# Autodesk Inventor assembly: OmniWheel
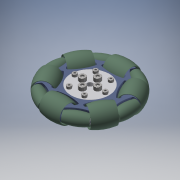
[picture p0: Inventor's stored thumbnail of the model, 180x180]
Saved by Autodesk Inventor 2019.1 (Build 231200000, 200)
## iProperties
Created: 2018-08-15
Part Number: OmniWheel
Material: Generisch
Document SubType Name: Assembly
Designer: JochenAlt
Author: JochenAlt
## Documents named in this file (9)
- D:\Projects\Ondine\CAD\OmniWheel.iam
- D:\Projects\Ondine\CAD\OmniWheel.ipt
- D:\Projects\Ondine\CAD\Mounting Hub.ipt
- C:\Users\JochenAlt\Documents\Inventor\Content Center Files\R2019\de-DE\DIN 912\DIN 912 - M3 x 0,5 x 8 x 6,75.ipt
- C:\Users\JochenAlt\Documents\Inventor\Content Center Files\R2019\de-DE\DIN 912\DIN 912 - M2 x 0,4 x 8 x 7.ipt
- C:\Users\JochenAlt\Documents\Inventor\Content Center Files\R2019\de-DE\DIN 934\DIN 934 - M2 x 0,4.ipt
- D:\Projects\Ondine\CAD\OmniWheelAxisSmall.ipt
- D:\Projects\Ondine\CAD\OmniWheelAxisBig.ipt
- D:\Projects\Ondine\CAD\Bearings\W 618_2 X.iam
## Components (54 placed, 8 different names)
1. OmniWheel:1 — Passend:1, Passend:2, Einfügen:1, Einfügen:2, Einfügen:3, Einfügen:4, Einfügen:5, Einfügen:6, Einfügen:7, Einfügen:8, Einfügen:9, Einfügen:10, Passend:4, Passend:6, Passend:8, Passend:10, Passend:12, Passend:14, Passend:15, Passend:16, Passend:17, Passend:18, Passend:19, Passend:20, Passend:21, Passend:23, Passend:24, Passend:25, Passend:26, Passend:27, Passend:28, Passend:29, Passend:30, Passend:31, Passend:32, Passend:33, Passend:34, Passend:35, Passend:36, Passend:37, Passend:38, Passend:39, Passend:64, Passend:65, Passend:66, Passend:67, Passend:68, Passend:69, Passend:70, Passend:71, Passend:72, Passend:73, Passend:74, Passend:75, Passend:76, Passend:77, Passend:78, Passend:79, Passend:80, Passend:81, Passend:82, Passend:83, Passend:84, Passend:85, Passend:86, Passend:87
2. Mounting Hub:1 — Passend:1, Passend:2
3. OmniWheelAxisSmall:1 — Passend:23, Passend:36, Passend:54, Passend:55
4. OmniWheelAxisSmall:2 — Passend:24, Passend:35, Passend:52, Passend:53
5. OmniWheelAxisSmall:3 — Passend:26, Passend:38, Passend:42, Passend:43
6. OmniWheelAxisSmall:4 — Passend:27, Passend:28, Passend:58, Passend:59
7. OmniWheelAxisSmall:5 — Passend:25, Passend:39, Passend:46, Passend:47
8. OmniWheelAxisSmall:6 — Passend:21, Passend:37, Passend:62, Passend:63
9. OmniWheelAxisBig:1 — Passend:15, Passend:31, Passend:60, Passend:61
10. OmniWheelAxisBig:2 — Passend:16, Passend:29, Passend:56, Passend:57
11. OmniWheelAxisBig:3 — Passend:19, Passend:33, Passend:44, Passend:45
12. OmniWheelAxisBig:4 — Passend:20, Passend:32, Passend:40, Passend:41
13. OmniWheelAxisBig:5 — Passend:17, Passend:30, Passend:50, Passend:51
14. OmniWheelAxisBig:6 — Passend:18, Passend:34, Passend:48, Passend:49
15. DIN 912 - ersetzt durch DIN EN ISO 4762 M3 x 8:1 — Einfügen:1
16. DIN 912 - ersetzt durch DIN EN ISO 4762 M3 x 8:2 — Einfügen:2
17. DIN 912 - ersetzt durch DIN EN ISO 4762 M3 x 8:3 — Einfügen:3
18. DIN 912 - ersetzt durch DIN EN ISO 4762 M3 x 8:4 — Einfügen:4
19. DIN 912 - ersetzt durch DIN EN ISO 4762 M2 x 8:1 — Einfügen:5, Passend:13
20. DIN 912 - ersetzt durch DIN EN ISO 4762 M2 x 8:2 — Einfügen:6, Passend:9
21. DIN 912 - ersetzt durch DIN EN ISO 4762 M2 x 8:3 — Einfügen:7, Passend:7
22. DIN 912 - ersetzt durch DIN EN ISO 4762 M2 x 8:4 — Einfügen:8, Passend:5
23. DIN 912 - ersetzt durch DIN EN ISO 4762 M2 x 8:5 — Einfügen:9, Passend:11
24. DIN 912 - ersetzt durch DIN EN ISO 4762 M2 x 8:6 — Einfügen:10, Passend:3
25. DIN 934 - ersetzt durch DIN EN 24032/28673/28674 M2:1 — Passend:3, Passend:4
26. DIN 934 - ersetzt durch DIN EN 24032/28673/28674 M2:2 — Passend:5, Passend:6
27. DIN 934 - ersetzt durch DIN EN 24032/28673/28674 M2:3 — Passend:7, Passend:8
28. DIN 934 - ersetzt durch DIN EN 24032/28673/28674 M2:4 — Passend:9, Passend:10
29. DIN 934 - ersetzt durch DIN EN 24032/28673/28674 M2:5 — Passend:11, Passend:12
30. DIN 934 - ersetzt durch DIN EN 24032/28673/28674 M2:6 — Passend:13, Passend:14
31. W 618_2 X:1 [sub-assembly] — Passend:41, Passend:64
32. W 618_2 X:2 [sub-assembly] — Passend:42, Passend:87
33. W 618_2 X:3 [sub-assembly] — Passend:40, Passend:65
34. W 618_2 X:4 [sub-assembly] — Passend:43, Passend:86
35. W 618_2 X:5 [sub-assembly] — Passend:44, Passend:85
36. W 618_2 X:6 [sub-assembly] — Passend:59, Passend:70
37. W 618_2 X:7 [sub-assembly] — Passend:58, Passend:71
38. W 618_2 X:8 [sub-assembly] — Passend:53, Passend:81
39. W 618_2 X:9 [sub-assembly] — Passend:52, Passend:80
40. W 618_2 X:10 [sub-assembly] — Passend:57, Passend:72
41. W 618_2 X:11 [sub-assembly] — Passend:51, Passend:76
42. W 618_2 X:12 [sub-assembly] — Passend:50, Passend:77
43. W 618_2 X:13 [sub-assembly] — Passend:54, Passend:75
44. W 618_2 X:14 [sub-assembly] — Passend:48, Passend:78
45. W 618_2 X:15 [sub-assembly] — Passend:49, Passend:79
46. W 618_2 X:16 [sub-assembly] — Passend:55, Passend:74
47. W 618_2 X:17 [sub-assembly] — Passend:56, Passend:73
48. W 618_2 X:18 [sub-assembly] — Passend:45, Passend:84
49. W 618_2 X:19 [sub-assembly] — Passend:46, Passend:82
50. W 618_2 X:20 [sub-assembly] — Passend:47, Passend:83
51. W 618_2 X:21 [sub-assembly] — Passend:60, Passend:69
52. W 618_2 X:22 [sub-assembly] — Passend:63, Passend:66
53. W 618_2 X:23 [sub-assembly] — Passend:62, Passend:67
54. W 618_2 X:24 [sub-assembly] — Passend:61, Passend:68
## Relationships (96: Mate 86, Insert 10)
- Passend:1 [Mate]: OmniWheel:1 ↔ Mounting Hub:1
- Passend:2 [Mate]: OmniWheel:1 ↔ Mounting Hub:1
- Einfügen:1 [Insert]: OmniWheel:1 ↔ DIN 912 - ersetzt durch DIN EN ISO 4762 M3 x 8:1
- Einfügen:2 [Insert]: OmniWheel:1 ↔ DIN 912 - ersetzt durch DIN EN ISO 4762 M3 x 8:2
- Einfügen:3 [Insert]: OmniWheel:1 ↔ DIN 912 - ersetzt durch DIN EN ISO 4762 M3 x 8:3
- Einfügen:4 [Insert]: OmniWheel:1 ↔ DIN 912 - ersetzt durch DIN EN ISO 4762 M3 x 8:4
- Einfügen:5 [Insert]: OmniWheel:1 ↔ DIN 912 - ersetzt durch DIN EN ISO 4762 M2 x 8:1
- Einfügen:6 [Insert]: OmniWheel:1 ↔ DIN 912 - ersetzt durch DIN EN ISO 4762 M2 x 8:2
- Einfügen:7 [Insert]: OmniWheel:1 ↔ DIN 912 - ersetzt durch DIN EN ISO 4762 M2 x 8:3
- Einfügen:8 [Insert]: OmniWheel:1 ↔ DIN 912 - ersetzt durch DIN EN ISO 4762 M2 x 8:4
- Einfügen:9 [Insert]: OmniWheel:1 ↔ DIN 912 - ersetzt durch DIN EN ISO 4762 M2 x 8:5
- Einfügen:10 [Insert]: OmniWheel:1 ↔ DIN 912 - ersetzt durch DIN EN ISO 4762 M2 x 8:6
- Passend:3 [Mate]: DIN 912 - ersetzt durch DIN EN ISO 4762 M2 x 8:6 ↔ DIN 934 - ersetzt durch DIN EN 24032/28673/28674 M2:1
- Passend:4 [Mate]: OmniWheel:1 ↔ DIN 934 - ersetzt durch DIN EN 24032/28673/28674 M2:1
- Passend:5 [Mate]: DIN 912 - ersetzt durch DIN EN ISO 4762 M2 x 8:4 ↔ DIN 934 - ersetzt durch DIN EN 24032/28673/28674 M2:2
- Passend:6 [Mate]: OmniWheel:1 ↔ DIN 934 - ersetzt durch DIN EN 24032/28673/28674 M2:2
- Passend:7 [Mate]: DIN 912 - ersetzt durch DIN EN ISO 4762 M2 x 8:3 ↔ DIN 934 - ersetzt durch DIN EN 24032/28673/28674 M2:3
- Passend:8 [Mate]: OmniWheel:1 ↔ DIN 934 - ersetzt durch DIN EN 24032/28673/28674 M2:3
- Passend:9 [Mate]: DIN 912 - ersetzt durch DIN EN ISO 4762 M2 x 8:2 ↔ DIN 934 - ersetzt durch DIN EN 24032/28673/28674 M2:4
- Passend:10 [Mate]: OmniWheel:1 ↔ DIN 934 - ersetzt durch DIN EN 24032/28673/28674 M2:4
- Passend:11 [Mate]: DIN 912 - ersetzt durch DIN EN ISO 4762 M2 x 8:5 ↔ DIN 934 - ersetzt durch DIN EN 24032/28673/28674 M2:5
- Passend:12 [Mate]: OmniWheel:1 ↔ DIN 934 - ersetzt durch DIN EN 24032/28673/28674 M2:5
- Passend:13 [Mate]: DIN 912 - ersetzt durch DIN EN ISO 4762 M2 x 8:1 ↔ DIN 934 - ersetzt durch DIN EN 24032/28673/28674 M2:6
- Passend:14 [Mate]: OmniWheel:1 ↔ DIN 934 - ersetzt durch DIN EN 24032/28673/28674 M2:6
- Passend:15 [Mate]: OmniWheel:1 ↔ OmniWheelAxisBig:1
- Passend:16 [Mate]: OmniWheel:1 ↔ OmniWheelAxisBig:2
- Passend:17 [Mate]: OmniWheel:1 ↔ OmniWheelAxisBig:5
- Passend:18 [Mate]: OmniWheel:1 ↔ OmniWheelAxisBig:6
- Passend:19 [Mate]: OmniWheel:1 ↔ OmniWheelAxisBig:3
- Passend:20 [Mate]: OmniWheel:1 ↔ OmniWheelAxisBig:4
- Passend:21 [Mate]: OmniWheel:1 ↔ OmniWheelAxisSmall:6
- Passend:23 [Mate]: OmniWheel:1 ↔ OmniWheelAxisSmall:1
- Passend:24 [Mate]: OmniWheel:1 ↔ OmniWheelAxisSmall:2
- Passend:25 [Mate]: OmniWheel:1 ↔ OmniWheelAxisSmall:5
- Passend:26 [Mate]: OmniWheel:1 ↔ OmniWheelAxisSmall:3
- Passend:27 [Mate]: OmniWheel:1 ↔ OmniWheelAxisSmall:4
- Passend:28 [Mate]: OmniWheel:1 ↔ OmniWheelAxisSmall:4
- Passend:29 [Mate] (-2 mm): OmniWheel:1 ↔ OmniWheelAxisBig:2
- Passend:30 [Mate] (2 mm): OmniWheel:1 ↔ OmniWheelAxisBig:5
- Passend:31 [Mate] (2 mm): OmniWheel:1 ↔ OmniWheelAxisBig:1
- Passend:32 [Mate] (2 mm): OmniWheel:1 ↔ OmniWheelAxisBig:4
- Passend:33 [Mate] (2 mm): OmniWheel:1 ↔ OmniWheelAxisBig:3
- Passend:34 [Mate] (2 mm): OmniWheel:1 ↔ OmniWheelAxisBig:6
- Passend:35 [Mate]: OmniWheel:1 ↔ OmniWheelAxisSmall:2
- Passend:36 [Mate]: OmniWheel:1 ↔ OmniWheelAxisSmall:1
- Passend:37 [Mate]: OmniWheel:1 ↔ OmniWheelAxisSmall:6
- Passend:38 [Mate]: OmniWheel:1 ↔ OmniWheelAxisSmall:3
- Passend:39 [Mate]: OmniWheel:1 ↔ OmniWheelAxisSmall:5
- Passend:40 [Mate]: OmniWheelAxisBig:4 ↔ W 618_2 X:3
- Passend:41 [Mate]: OmniWheelAxisBig:4 ↔ W 618_2 X:1
- Passend:42 [Mate]: OmniWheelAxisSmall:3 ↔ W 618_2 X:2
- Passend:43 [Mate]: OmniWheelAxisSmall:3 ↔ W 618_2 X:4
- Passend:44 [Mate]: OmniWheelAxisBig:3 ↔ W 618_2 X:5
- Passend:45 [Mate]: OmniWheelAxisBig:3 ↔ W 618_2 X:18
- Passend:46 [Mate]: OmniWheelAxisSmall:5 ↔ W 618_2 X:19
- Passend:47 [Mate]: OmniWheelAxisSmall:5 ↔ W 618_2 X:20
- Passend:48 [Mate]: OmniWheelAxisBig:6 ↔ W 618_2 X:14
- Passend:49 [Mate]: OmniWheelAxisBig:6 ↔ W 618_2 X:15
- Passend:50 [Mate]: OmniWheelAxisBig:5 ↔ W 618_2 X:12
- Passend:51 [Mate]: OmniWheelAxisBig:5 ↔ W 618_2 X:11
- Passend:52 [Mate]: OmniWheelAxisSmall:2 ↔ W 618_2 X:9
- Passend:53 [Mate]: OmniWheelAxisSmall:2 ↔ W 618_2 X:8
- Passend:54 [Mate]: OmniWheelAxisSmall:1 ↔ W 618_2 X:13
- Passend:55 [Mate]: OmniWheelAxisSmall:1 ↔ W 618_2 X:16
- Passend:56 [Mate]: OmniWheelAxisBig:2 ↔ W 618_2 X:17
- Passend:57 [Mate]: OmniWheelAxisBig:2 ↔ W 618_2 X:10
- Passend:58 [Mate]: OmniWheelAxisSmall:4 ↔ W 618_2 X:7
- Passend:59 [Mate]: OmniWheelAxisSmall:4 ↔ W 618_2 X:6
- Passend:60 [Mate]: OmniWheelAxisBig:1 ↔ W 618_2 X:21
- Passend:61 [Mate]: OmniWheelAxisBig:1 ↔ W 618_2 X:24
- Passend:62 [Mate]: OmniWheelAxisSmall:6 ↔ W 618_2 X:23
- Passend:63 [Mate]: OmniWheelAxisSmall:6 ↔ W 618_2 X:22
- Passend:64 [Mate]: OmniWheel:1 ↔ W 618_2 X:1
- Passend:65 [Mate]: OmniWheel:1 ↔ W 618_2 X:3
- Passend:66 [Mate]: OmniWheel:1 ↔ W 618_2 X:22
- Passend:67 [Mate]: OmniWheel:1 ↔ W 618_2 X:23
- Passend:68 [Mate]: OmniWheel:1 ↔ W 618_2 X:24
- Passend:69 [Mate]: OmniWheel:1 ↔ W 618_2 X:21
- Passend:70 [Mate]: OmniWheel:1 ↔ W 618_2 X:6
- Passend:71 [Mate]: OmniWheel:1 ↔ W 618_2 X:7
- Passend:72 [Mate]: OmniWheel:1 ↔ W 618_2 X:10
- Passend:73 [Mate]: OmniWheel:1 ↔ W 618_2 X:17
- Passend:74 [Mate]: OmniWheel:1 ↔ W 618_2 X:16
- Passend:75 [Mate]: OmniWheel:1 ↔ W 618_2 X:13
- Passend:76 [Mate]: OmniWheel:1 ↔ W 618_2 X:11
- Passend:77 [Mate]: OmniWheel:1 ↔ W 618_2 X:12
- Passend:78 [Mate]: OmniWheel:1 ↔ W 618_2 X:14
- Passend:79 [Mate]: OmniWheel:1 ↔ W 618_2 X:15
- Passend:80 [Mate]: OmniWheel:1 ↔ W 618_2 X:9
- Passend:81 [Mate]: OmniWheel:1 ↔ W 618_2 X:8
- Passend:82 [Mate]: OmniWheel:1 ↔ W 618_2 X:19
- Passend:83 [Mate]: OmniWheel:1 ↔ W 618_2 X:20
- Passend:84 [Mate]: OmniWheel:1 ↔ W 618_2 X:18
- Passend:85 [Mate]: OmniWheel:1 ↔ W 618_2 X:5
- Passend:86 [Mate]: OmniWheel:1 ↔ W 618_2 X:4
- Passend:87 [Mate]: OmniWheel:1 ↔ W 618_2 X:2
